# Autodesk Inventor assembly: Assembly_Dumb
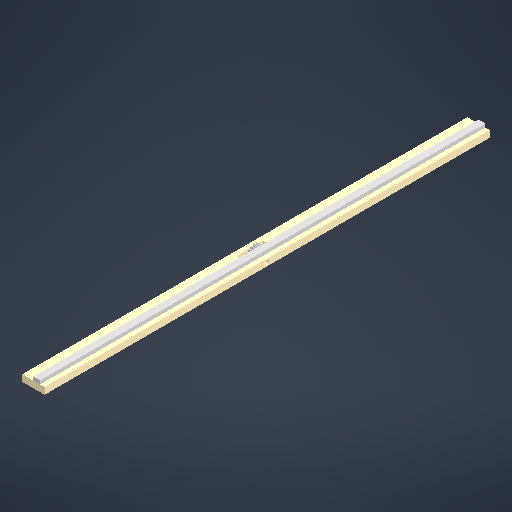
[picture p0: Inventor's stored thumbnail of the model, 512x512]
Saved by Autodesk Inventor 2026.1 (Build 301233020, 233B)
## iProperties
Created: 2026-03-11
Part Number: Assembly_Dumb
Document SubType Name: Assembly
Designer: elaij
Author: elaij
## Documents named in this file (4)
- C:\Users\elaij\OneDrive\Documents\MD Project 314\CAD_Concepts\Assembly_Dumb.iam
- C:\Users\elaij\OneDrive\Documents\MD Project 314\CAD_Concepts\Layer.ipt
- C:\Users\elaij\OneDrive\Documents\MD Project 314\CAD_Concepts\Rack.ipt
- C:\Users\elaij\OneDrive\Documents\MD Project 314\CAD_Concepts\Gear_Basic.ipt
## Components (3 placed, 3 different names)
1. Layer:1 — Mate:1, Flush:1, Mate:2, Mate:3, Mate:4
2. Rack:1 — Mate:1, Flush:1, Mate:4
3. Gear_Basic:1 — Mate:2, Mate:3, Angle:1
## Relationships (6: Mate 4, Flush 1, Angle 1)
- Mate:1: Layer:1 ↔ Rack:1
- Flush:1: Layer:1 ↔ Rack:1
- Mate:2: Layer:1 ↔ Gear_Basic:1
- Mate:3: Layer:1 ↔ Gear_Basic:1
- Mate:4: Layer:1 ↔ Rack:1
- Angle:1 (139 deg): Gear_Basic:1
